# Autodesk Inventor assembly: UBG-ChipKick
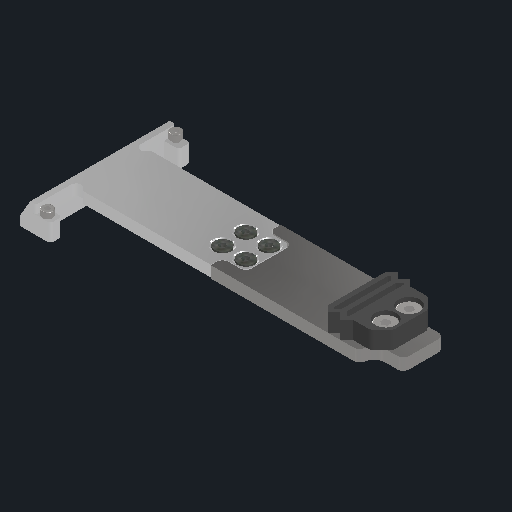
[picture p0: Inventor's stored thumbnail of the model, 512x512]
Saved by Autodesk Inventor 2025.2 (Build 292293000, 293)
## iProperties
Created: 2024-11-08
Part Number: UBG-ChipKick
Document SubType Name: Assembly
Designer: Fabian
Author: Fabian
## Documents named in this file (7)
- C:\Users\Faabs\Desktop\HBG v2025\Unterbaugruppen\UBG-Schussbauteile\UBG-Hochschuss\UBG-Hochschuss.iam
- C:\Users\Faabs\Desktop\HBG v2025\Unterbaugruppen\UBG-Schussbauteile\UBG-Hochschuss\Bauteile\Tauchkern.ipt
- C:\Users\Faabs\Desktop\HBG v2025\Unterbaugruppen\UBG-Schussbauteile\UBG-Schuss\Bauteile\SchussEisen.ipt
- C:\Users\Faabs\Desktop\HBG v2025\Verbindungselemente\ISO 10642\ISO 10642  - M3  x  4.ipt
- C:\Users\Faabs\Desktop\HBG v2025\Verbindungselemente\DIN 912\DIN 912 - M2 x 0,4 x 6 x 5.ipt
- C:\Users\Faabs\Desktop\HBG v2025\Unterbaugruppen\UBG-Schussbauteile\UBG-Schuss\Bauteile\SchussDämpfung.ipt
- C:\Users\Faabs\Desktop\HBG v2025\Verbindungselemente\DIN 7984\DIN 7984 - M4 x 6.ipt
## Components (11 placed, 6 different names)
1. Tauchkern:1 — Passend:3, Passend:4, Fluchtend:4, Einfügen:10, Einfügen:11, Einfügen:12, Einfügen:15, Einfügen:16
2. SchussEisen:1 — Passend:1, Fluchtend:3, Passend:2, Passend:3, Passend:4, Fluchtend:4, Einfügen:9, Einfügen:13, Einfügen:14
3. SchussDämpfung:1 — Einfügen:7, Einfügen:8, Einfügen:13, Einfügen:14
4. DIN EN ISO 10642 M3  x  8:1 — Einfügen:10
5. DIN EN ISO 10642 M3  x  8:2 — Einfügen:11
6. DIN EN ISO 10642 M3  x  8:3 — Einfügen:12
7. DIN EN ISO 10642 M3  x  8:4 — Einfügen:9
8. DIN 912 - ersetzt durch DIN EN ISO 4762 M2 x 6:1 — Einfügen:16
9. DIN 912 - ersetzt durch DIN EN ISO 4762 M2 x 6:2 — Einfügen:15
10. DIN 7984 M4 x 6:1 — Einfügen:7
11. DIN 7984 M4 x 6:2 — Einfügen:8
## Relationships (16: Insert 10, Mate 4, Flush 2)
- Einfügen:7 [Insert]: SchussDämpfung:1 ↔ DIN 7984 M4 x 6:1
- Einfügen:8 [Insert]: SchussDämpfung:1 ↔ DIN 7984 M4 x 6:2
- Passend:1 [Mate]: SchussEisen:1
- Fluchtend:3 [Flush]: SchussEisen:1
- Passend:2 [Mate]: SchussEisen:1
- Passend:3 [Mate]: Tauchkern:1 ↔ SchussEisen:1
- Passend:4 [Mate]: Tauchkern:1 ↔ SchussEisen:1
- Fluchtend:4 [Flush] (0.1 mm): Tauchkern:1 ↔ SchussEisen:1
- Einfügen:9 [Insert]: SchussEisen:1 ↔ DIN EN ISO 10642 M3  x  8:4
- Einfügen:10 [Insert]: Tauchkern:1 ↔ DIN EN ISO 10642 M3  x  8:1
- Einfügen:11 [Insert]: Tauchkern:1 ↔ DIN EN ISO 10642 M3  x  8:2
- Einfügen:12 [Insert]: Tauchkern:1 ↔ DIN EN ISO 10642 M3  x  8:3
- Einfügen:13 [Insert]: SchussEisen:1 ↔ SchussDämpfung:1
- Einfügen:14 [Insert]: SchussEisen:1 ↔ SchussDämpfung:1
- Einfügen:15 [Insert] (1 mm): Tauchkern:1 ↔ DIN 912 - ersetzt durch DIN EN ISO 4762 M2 x 6:2
- Einfügen:16 [Insert]: Tauchkern:1 ↔ DIN 912 - ersetzt durch DIN EN ISO 4762 M2 x 6:1
